# Autodesk Inventor assembly: mini-pakiet-12sp1
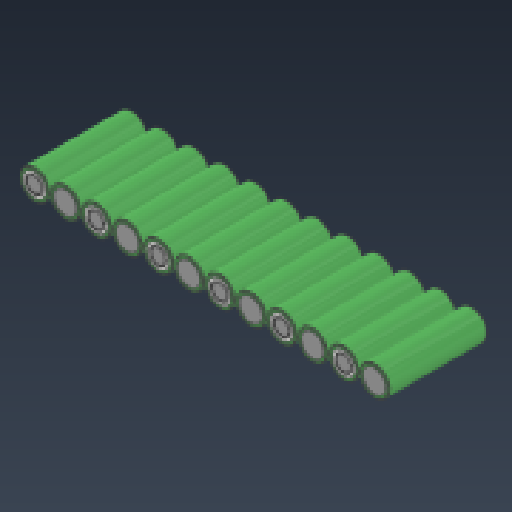
[picture p0: Inventor's stored thumbnail of the model, 512x512]
Saved by Autodesk Inventor 2023 (Build 270158000, 158)
## iProperties
Created: 2025-11-13
Part Number: mini-pakiet-12sp1
Document SubType Name: Assembly
Designer: szymo
Author: szymo
## Documents named in this file (2)
- D:\tech\diy\e-skateboard\projekcik-inventor\mini-pakiet-12sp1.iam
- D:\tech\diy\e-skateboard\projekcik-inventor\21700.ipt
## Components (12 placed, 1 different names)
1. 21700:1 — Tangent:1, Flush:1, Tangent:13
2. 21700:2 — Flush:1, Flush:2, Tangent:12, Tangent:13, Tangent:14
3. 21700:3 — Tangent:2, Flush:2, Flush:3, Tangent:14, Tangent:15
4. 21700:4 — Tangent:3, Flush:3, Flush:4, Tangent:15, Tangent:16
5. 21700:5 — Tangent:4, Flush:4, Flush:5, Tangent:16, Tangent:17
6. 21700:6 — Tangent:5, Flush:5, Flush:6, Tangent:17, Tangent:18
7. 21700:7 — Tangent:6, Flush:6, Flush:7, Tangent:18, Tangent:19
8. 21700:8 — Tangent:7, Flush:7, Flush:8, Tangent:19, Tangent:20
9. 21700:9 — Tangent:8, Flush:8, Flush:9, Tangent:20, Tangent:21
10. 21700:10 — Tangent:9, Flush:9, Flush:10, Tangent:21, Tangent:22
11. 21700:11 — Tangent:10, Flush:10, Flush:11, Tangent:22, Tangent:23
12. 21700:12 — Tangent:11, Flush:11, Tangent:23
## Relationships (34: Tangent 23, Flush 11)
- Tangent:1: 21700:1
- Flush:1: 21700:1 ↔ 21700:2
- Tangent:2: 21700:3
- Tangent:3: 21700:4
- Tangent:4: 21700:5
- Tangent:5: 21700:6
- Tangent:6: 21700:7
- Tangent:7: 21700:8
- Tangent:8: 21700:9
- Tangent:9: 21700:10
- Tangent:10: 21700:11
- Tangent:11: 21700:12
- Flush:2: 21700:2 ↔ 21700:3
- Flush:3: 21700:3 ↔ 21700:4
- Flush:4: 21700:4 ↔ 21700:5
- Flush:5: 21700:5 ↔ 21700:6
- Flush:6: 21700:6 ↔ 21700:7
- Flush:7: 21700:7 ↔ 21700:8
- Flush:8: 21700:8 ↔ 21700:9
- Flush:9: 21700:9 ↔ 21700:10
- Flush:10: 21700:10 ↔ 21700:11
- Flush:11: 21700:11 ↔ 21700:12
- Tangent:12: 21700:2
- Tangent:13 (1 mm): 21700:1 ↔ 21700:2
- Tangent:14 (1 mm): 21700:2 ↔ 21700:3
- Tangent:15 (1 mm): 21700:3 ↔ 21700:4
- Tangent:16 (1 mm): 21700:4 ↔ 21700:5
- Tangent:17 (1 mm): 21700:5 ↔ 21700:6
- Tangent:18 (1 mm): 21700:6 ↔ 21700:7
- Tangent:19 (1 mm): 21700:7 ↔ 21700:8
- Tangent:20 (1 mm): 21700:8 ↔ 21700:9
- Tangent:21 (1 mm): 21700:9 ↔ 21700:10
- Tangent:22 (1 mm): 21700:10 ↔ 21700:11
- Tangent:23 (1 mm): 21700:11 ↔ 21700:12
## Named parameters: batteries_offset = 1 mm
